# Autodesk Inventor assembly: assembly_orbiter
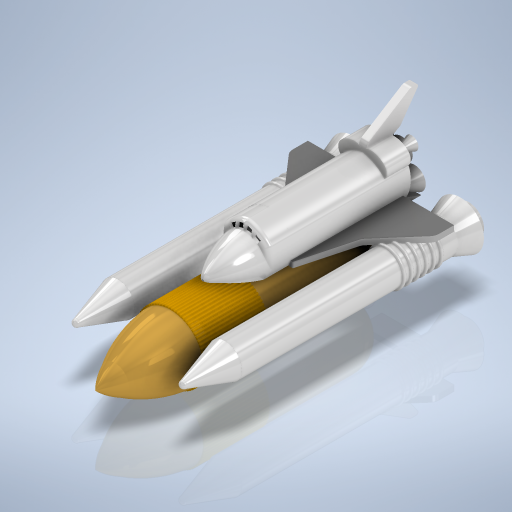
[picture p0: Inventor's stored thumbnail of the model, 512x512]
Saved by Autodesk Inventor 2024 (Build 280153000, 153)
## iProperties
Created: 2023-06-07
Part Number: assembly_orbiter
Document SubType Name: Assembly
Designer: tamiz
Author: tamiz
## Documents named in this file (13)
- C:\Users\tamiz\Documents\IITGN\Summer Term\EG\Project\Designs\assembly_orbiter.iam
- C:\Users\tamiz\Documents\IITGN\Summer Term\EG\Project\Designs\cabin_crew.ipt
- C:\Users\tamiz\Documents\IITGN\Summer Term\EG\Project\Designs\body.ipt
- C:\Users\tamiz\Documents\IITGN\Summer Term\EG\Project\Designs\nose.ipt
- C:\Users\tamiz\Documents\IITGN\Summer Term\EG\Project\Designs\engines.ipt
- C:\Users\tamiz\Documents\IITGN\Summer Term\EG\Project\Designs\wings.ipt
- C:\Users\tamiz\Documents\IITGN\Summer Term\EG\Project\Designs\vertical_tail.ipt
- C:\Users\tamiz\Documents\IITGN\Summer Term\EG\Project\Designs\body_flaps.ipt
- C:\Users\tamiz\Documents\IITGN\Summer Term\EG\Project\Designs\srb_body.ipt
- C:\Users\tamiz\Documents\IITGN\Summer Term\EG\Project\Designs\srb_thrusters_and_vectors.ipt
- C:\Users\tamiz\Documents\IITGN\Summer Term\EG\Project\Designs\ex_tank_H.ipt
- C:\Users\tamiz\Documents\IITGN\Summer Term\EG\Project\Designs\ex_tank_inter.ipt
- C:\Users\tamiz\Documents\IITGN\Summer Term\EG\Project\Designs\ex_tank_O.ipt
## Components (14 placed, 12 different names)
1. cabin_crew:1 — Mate:1, Insert:1, Mate:2
2. body:1 — Mate:1, Insert:1, Mate:3, Mate:4, Mate:5, Flush:1, Flush:2
3. nose:1 — Mate:2
4. engines:1 — Mate:3, Mate:4, Mate:5, Mate:6, Flush:3, Mate:7, Mate:8, Flush:4, Flush:5
5. wings:1 — Flush:1, Flush:2
6. vertical_tail:1 — Mate:6, Flush:3
7. body_flaps:1 — Mate:7, Mate:8
8. srb_body:1 — Flush:5, Mate:9
9. srb_body:2 — Flush:4, Mate:10, Mate:11
10. srb_thrusters_and_vectors:1 — Mate:10, Mate:11
11. srb_thrusters_and_vectors:2 — Mate:9
12. ex_tank_H:1 — Rotational:1
13. ex_tank_inter:1 — Rotational:1, Rotational:2
14. ex_tank_O:1 — Rotational:2
## Relationships (19: Mate 11, Flush 5, RevoluteJoint 2, Insert 1)
- Mate:1: cabin_crew:1 ↔ body:1
- Insert:1: cabin_crew:1 ↔ body:1
- Mate:2: cabin_crew:1 ↔ nose:1
- Mate:3: body:1 ↔ engines:1
- Mate:4: body:1 ↔ engines:1
- Mate:5: body:1 ↔ engines:1
- Flush:1: body:1 ↔ wings:1
- Flush:2: body:1 ↔ wings:1
- Mate:6: engines:1 ↔ vertical_tail:1
- Flush:3: engines:1 ↔ vertical_tail:1
- Mate:7: engines:1 ↔ body_flaps:1
- Mate:8: engines:1 ↔ body_flaps:1
- Flush:4: engines:1 ↔ srb_body:2
- Flush:5: engines:1 ↔ srb_body:1
- Mate:9: srb_body:1 ↔ srb_thrusters_and_vectors:2
- Mate:10: srb_body:2 ↔ srb_thrusters_and_vectors:1
- Mate:11: srb_body:2 ↔ srb_thrusters_and_vectors:1
- Rotational:1 [RevoluteJoint]: ex_tank_H:1 ↔ ex_tank_inter:1
- Rotational:2 [RevoluteJoint]: ex_tank_inter:1 ↔ ex_tank_O:1
